# Autodesk Inventor assembly: ConnectorAssembly
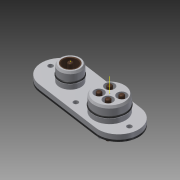
[picture p0: Inventor's stored thumbnail of the model, 180x180]
Saved by Autodesk Inventor 2014 SP2 (Build 180246200, 246)
## iProperties
Created: 2015-09-20
Part Number: ConnectorAssembly
Document SubType Name: Assembly
Designer: Lukasz Szmit
Author: Lukasz Szmit
## Documents named in this file (7)
- H:\Documents\Projects\mb\Ignition Module\Case\ConnectorAssembly.iam
- H:\Documents\Projects\mb\Ignition Module\Case\Connector.ipt
- H:\Documents\Projects\mb\Ignition Module\Case\ConnectorPin.ipt
- H:\Documents\Projects\mb\Ignition Module\Case\ConnectorSeal.ipt
- H:\Documents\Projects\mb\Ignition Module\Case\ConnectorSocket.ipt
- H:\Documents\Projects\mb\Ignition Module\Case\OringBig.ipt
- H:\Documents\Projects\mb\Ignition Module\Case\OringSmall.ipt
## Components (10 placed, 6 different names)
1. Connector:1 — Symmetry:1, Symmetry:2, Mate:1, Symmetry:4, Tangent:1, Symmetry:5, Tangent:2, Symmetry:6, Mate:3, Insert:1, Insert:2, Insert:3, Insert:4, Mate:4, Tangent:3, Tangent:4
2. ConnectorPin:1 — Insert:4
3. ConnectorSeal:1 — Mate:4, Tangent:3, Tangent:4
4. ConnectorSocket:1 — Symmetry:2, Mate:1
5. OringBig:1 — Symmetry:4, Tangent:1
6. OringSmall:1 — Symmetry:5, Tangent:2
7. ConnectorPin:2 — Insert:1
8. ConnectorPin:3 — Insert:3
9. ConnectorPin:4 — Insert:2
10. ConnectorPin:5 — Symmetry:6, Mate:3
## Relationships (16: Symmetry 5, Tangent 4, Insert 4, Mate 3)
- Symmetry:1: Connector:1
- Symmetry:2: Connector:1 ↔ ConnectorSocket:1
- Mate:1: Connector:1 ↔ ConnectorSocket:1
- Symmetry:4: Connector:1 ↔ OringBig:1
- Tangent:1: Connector:1 ↔ OringBig:1
- Symmetry:5: Connector:1 ↔ OringSmall:1
- Tangent:2: Connector:1 ↔ OringSmall:1
- Symmetry:6: Connector:1 ↔ ConnectorPin:5
- Mate:3: Connector:1 ↔ ConnectorPin:5
- Insert:1 (-13.5 mm): Connector:1 ↔ ConnectorPin:2
- Insert:2 (-13.5 mm): Connector:1 ↔ ConnectorPin:4
- Insert:3 (-13.5 mm): Connector:1 ↔ ConnectorPin:3
- Insert:4 (-13.5 mm): Connector:1 ↔ ConnectorPin:1
- Mate:4: Connector:1 ↔ ConnectorSeal:1
- Tangent:3: Connector:1 ↔ ConnectorSeal:1
- Tangent:4: Connector:1 ↔ ConnectorSeal:1
